# Autodesk Inventor assembly: 1000_Planar Winding Jig Overall Assembly_V1
(part 2 of 2)
- Mate:124: 1322_Clamp Holder_V1:2 ↔ 1323_Clamp Holder Pin_V1:2
- Mate:125: 1322_Clamp Holder_V1:1 ↔ 1323_Clamp Holder Pin_V1:1
- Angle:9 (0 deg): frame_1385mm:4 ↔ 1313_Former Bottom_V1:1
- Flush:135 (45 mm): 1324_Clamp Rail_V1:2 ↔ 1322_Clamp Holder_V1:2
- [Flush] (45 mm): 1324_Clamp Rail_V1:3 ↔ 1322_Clamp Holder_V1:3
- [Mate] (0.5 mm): 1324_Clamp Rail_V1:4 ↔ 1322_Clamp Holder_V1:3
- [Mate]: 1322_Clamp Holder_V1:3 ↔ 1321_Toggle Clamp_V1:3
- [Flush]: 1322_Clamp Holder_V1:3 ↔ 1321_Toggle Clamp_V1:3
- [Flush] (3 mm): 1322_Clamp Holder_V1:3 ↔ 1321_Toggle Clamp_V1:3
- [Mate]: 1322_Clamp Holder_V1:3 ↔ BS 3692 Precision hexagon bolts and screws (Full Threaded) - Metric M4 x 9:10
- [Mate]: 1322_Clamp Holder_V1:3 ↔ BS 3692 Precision hexagon bolts and screws (Full Threaded) - Metric M4 x 9:10
- [Angle] (0 deg): 1322_Clamp Holder_V1:3 ↔ BS 3692 Precision hexagon bolts and screws (Full Threaded) - Metric M4 x 9:10
- [Mate]: 1322_Clamp Holder_V1:3 ↔ BS 3692 Precision hexagon bolts and screws (Full Threaded) - Metric M4 x 9:9
- [Mate]: 1322_Clamp Holder_V1:3 ↔ BS 3692 Precision hexagon bolts and screws (Full Threaded) - Metric M4 x 9:9
- [Angle] (0 deg): 1322_Clamp Holder_V1:3 ↔ BS 3692 Precision hexagon bolts and screws (Full Threaded) - Metric M4 x 9:9
- [Flush]: BS 3692 Precision hexagon bolts and screws (Full Threaded) - Metric M4 x 9:11 ↔ BS 3692 Precision hexagon bolts and screws (Full Threaded) - Metric M4 x 9:12
- [Mate]: 1322_Clamp Holder_V1:3 ↔ BS 3692 Precision hexagon bolts and screws (Full Threaded) - Metric M4 x 9:12
- [Mate]: 1322_Clamp Holder_V1:3 ↔ BS 3692 Precision hexagon bolts and screws (Full Threaded) - Metric M4 x 9:12
- [Flush]: BS 3692 Precision hexagon bolts and screws (Full Threaded) - Metric M4 x 9:9 ↔ BS 3692 Precision hexagon bolts and screws (Full Threaded) - Metric M4 x 9:12
- [Mate]: 1322_Clamp Holder_V1:3 ↔ BS 3692 Precision hexagon bolts and screws (Full Threaded) - Metric M4 x 9:11
- [Flush]: BS 3692 Precision hexagon bolts and screws (Full Threaded) - Metric M4 x 9:10 ↔ BS 3692 Precision hexagon bolts and screws (Full Threaded) - Metric M4 x 9:11
- [Mate]: BS 3692 Precision hexagon bolts and screws (Full Threaded) - Metric M4 x 9:9 ↔ AS 1474 - Metric M4:9
- [Mate]: 1321_Toggle Clamp_V1:3 ↔ AS 1474 - Metric M4:9
- [Flush]: AS 1474 - Metric M4:10 ↔ AS 1474 - Metric M4:12
- [Flush]: AS 1474 - Metric M4:11 ↔ AS 1474 - Metric M4:12
- [Flush]: AS 1474 - Metric M4:10 ↔ AS 1474 - Metric M4:11
- [Mate]: BS 3692 Precision hexagon bolts and screws (Full Threaded) - Metric M4 x 9:12 ↔ AS 1474 - Metric M4:10
- [Mate]: 1321_Toggle Clamp_V1:3 ↔ AS 1474 - Metric M4:10
- [Mate]: BS 3692 Precision hexagon bolts and screws (Full Threaded) - Metric M4 x 9:11 ↔ AS 1474 - Metric M4:11
- [Mate]: 1321_Toggle Clamp_V1:3 ↔ AS 1474 - Metric M4:12
- [Mate]: BS 3692 Precision hexagon bolts and screws (Full Threaded) - Metric M4 x 9:10 ↔ AS 1474 - Metric M4:12
- [Flush]: AS 1474 - Metric M4:9 ↔ AS 1474 - Metric M4:12
- [Mate]: 1322_Clamp Holder_V1:4 ↔ 1321_Toggle Clamp_V1:4
- [Flush]: 1322_Clamp Holder_V1:4 ↔ 1321_Toggle Clamp_V1:4
- [Flush] (3 mm): 1322_Clamp Holder_V1:4 ↔ 1321_Toggle Clamp_V1:4
- [Mate]: 1322_Clamp Holder_V1:4 ↔ BS 3692 Precision hexagon bolts and screws (Full Threaded) - Metric M4 x 9:14
- [Mate]: 1322_Clamp Holder_V1:4 ↔ BS 3692 Precision hexagon bolts and screws (Full Threaded) - Metric M4 x 9:14
- [Angle] (0 deg): 1322_Clamp Holder_V1:4 ↔ BS 3692 Precision hexagon bolts and screws (Full Threaded) - Metric M4 x 9:14
- [Mate]: 1322_Clamp Holder_V1:4 ↔ BS 3692 Precision hexagon bolts and screws (Full Threaded) - Metric M4 x 9:13
- [Mate]: 1322_Clamp Holder_V1:4 ↔ BS 3692 Precision hexagon bolts and screws (Full Threaded) - Metric M4 x 9:13
- [Angle] (0 deg): 1322_Clamp Holder_V1:4 ↔ BS 3692 Precision hexagon bolts and screws (Full Threaded) - Metric M4 x 9:13
- [Flush]: BS 3692 Precision hexagon bolts and screws (Full Threaded) - Metric M4 x 9:15 ↔ BS 3692 Precision hexagon bolts and screws (Full Threaded) - Metric M4 x 9:16
- [Mate]: 1322_Clamp Holder_V1:4 ↔ BS 3692 Precision hexagon bolts and screws (Full Threaded) - Metric M4 x 9:16
- [Mate]: 1322_Clamp Holder_V1:4 ↔ BS 3692 Precision hexagon bolts and screws (Full Threaded) - Metric M4 x 9:16
- [Flush]: BS 3692 Precision hexagon bolts and screws (Full Threaded) - Metric M4 x 9:13 ↔ BS 3692 Precision hexagon bolts and screws (Full Threaded) - Metric M4 x 9:16
- [Mate]: 1322_Clamp Holder_V1:4 ↔ BS 3692 Precision hexagon bolts and screws (Full Threaded) - Metric M4 x 9:15
- [Flush]: BS 3692 Precision hexagon bolts and screws (Full Threaded) - Metric M4 x 9:14 ↔ BS 3692 Precision hexagon bolts and screws (Full Threaded) - Metric M4 x 9:15
- [Mate]: BS 3692 Precision hexagon bolts and screws (Full Threaded) - Metric M4 x 9:13 ↔ AS 1474 - Metric M4:13
- [Mate]: 1321_Toggle Clamp_V1:4 ↔ AS 1474 - Metric M4:13
- [Flush]: AS 1474 - Metric M4:14 ↔ AS 1474 - Metric M4:16
- [Flush]: AS 1474 - Metric M4:15 ↔ AS 1474 - Metric M4:16
- [Flush]: AS 1474 - Metric M4:14 ↔ AS 1474 - Metric M4:15
- [Mate]: BS 3692 Precision hexagon bolts and screws (Full Threaded) - Metric M4 x 9:16 ↔ AS 1474 - Metric M4:14
- [Mate]: 1321_Toggle Clamp_V1:4 ↔ AS 1474 - Metric M4:14
- [Mate]: BS 3692 Precision hexagon bolts and screws (Full Threaded) - Metric M4 x 9:15 ↔ AS 1474 - Metric M4:15
- [Mate]: 1321_Toggle Clamp_V1:4 ↔ AS 1474 - Metric M4:16
- [Mate]: BS 3692 Precision hexagon bolts and screws (Full Threaded) - Metric M4 x 9:14 ↔ AS 1474 - Metric M4:16
- [Flush]: AS 1474 - Metric M4:13 ↔ AS 1474 - Metric M4:16
- [Mate]: 1324_Clamp Rail_V1:4 ↔ 1322_Clamp Holder_V1:4
- [Mate]: 1322_Clamp Holder_V1:4 ↔ 1323_Clamp Holder Pin_V1:4
- [Mate]: 1322_Clamp Holder_V1:3 ↔ 1323_Clamp Holder Pin_V1:3
- [Flush] (45 mm): 1324_Clamp Rail_V1:4 ↔ 1322_Clamp Holder_V1:4
- Mate:160: 1311_Former Top_V1:1 ↔ 1324_Clamp Rail_V1:3
- Flush:156: 1324_Clamp Rail_V1:3 ↔ 1324_Clamp Rail_V1:4
- Mate:161: 1324_Clamp Rail_V1:4 ↔ 1322_Clamp Holder_V1:3
- Flush:157: 1322_Clamp Holder_V1:3 ↔ 1322_Clamp Holder_V1:4
- Mate:162: 1324_Clamp Rail_V1:3 ↔ 1322_Clamp Holder_V1:4
- Mate:163: 1311_Former Top_V1:1 ↔ 1324_Clamp Rail_V1:4
- Mate:164: 1311_Former Top_V1:1 ↔ 1324_Clamp Rail_V1:4
- Flush:158: 1324_Clamp Rail_V1:3 ↔ 1324_Clamp Rail_V1:4
- Flush:159: 1323_Clamp Holder Pin_V1:3 ↔ 1323_Clamp Holder Pin_V1:4
- Flush:160: 1311_Former Top_V1:1 ↔ 1323_Clamp Holder Pin_V1:4
- [Flush] (45 mm): 1324_Clamp Rail_V1:5 ↔ 1322_Clamp Holder_V1:5
- [Mate] (0.5 mm): 1324_Clamp Rail_V1:6 ↔ 1322_Clamp Holder_V1:5
- [Mate]: 1322_Clamp Holder_V1:5 ↔ 1321_Toggle Clamp_V1:5
- [Flush]: 1322_Clamp Holder_V1:5 ↔ 1321_Toggle Clamp_V1:5
- [Flush] (3 mm): 1322_Clamp Holder_V1:5 ↔ 1321_Toggle Clamp_V1:5
- [Mate]: 1322_Clamp Holder_V1:5 ↔ BS 3692 Precision hexagon bolts and screws (Full Threaded) - Metric M4 x 9:18
- [Mate]: 1322_Clamp Holder_V1:5 ↔ BS 3692 Precision hexagon bolts and screws (Full Threaded) - Metric M4 x 9:18
- [Angle] (0 deg): 1322_Clamp Holder_V1:5 ↔ BS 3692 Precision hexagon bolts and screws (Full Threaded) - Metric M4 x 9:18
- [Mate]: 1322_Clamp Holder_V1:5 ↔ BS 3692 Precision hexagon bolts and screws (Full Threaded) - Metric M4 x 9:17
- [Mate]: 1322_Clamp Holder_V1:5 ↔ BS 3692 Precision hexagon bolts and screws (Full Threaded) - Metric M4 x 9:17
- [Angle] (0 deg): 1322_Clamp Holder_V1:5 ↔ BS 3692 Precision hexagon bolts and screws (Full Threaded) - Metric M4 x 9:17
- [Flush]: BS 3692 Precision hexagon bolts and screws (Full Threaded) - Metric M4 x 9:19 ↔ BS 3692 Precision hexagon bolts and screws (Full Threaded) - Metric M4 x 9:20
- [Mate]: 1322_Clamp Holder_V1:5 ↔ BS 3692 Precision hexagon bolts and screws (Full Threaded) - Metric M4 x 9:20
- [Mate]: 1322_Clamp Holder_V1:5 ↔ BS 3692 Precision hexagon bolts and screws (Full Threaded) - Metric M4 x 9:20
- [Flush]: BS 3692 Precision hexagon bolts and screws (Full Threaded) - Metric M4 x 9:17 ↔ BS 3692 Precision hexagon bolts and screws (Full Threaded) - Metric M4 x 9:20
- [Mate]: 1322_Clamp Holder_V1:5 ↔ BS 3692 Precision hexagon bolts and screws (Full Threaded) - Metric M4 x 9:19
- [Flush]: BS 3692 Precision hexagon bolts and screws (Full Threaded) - Metric M4 x 9:18 ↔ BS 3692 Precision hexagon bolts and screws (Full Threaded) - Metric M4 x 9:19
- [Mate]: BS 3692 Precision hexagon bolts and screws (Full Threaded) - Metric M4 x 9:17 ↔ AS 1474 - Metric M4:17
- [Mate]: 1321_Toggle Clamp_V1:5 ↔ AS 1474 - Metric M4:17
- [Flush]: AS 1474 - Metric M4:18 ↔ AS 1474 - Metric M4:20
- [Flush]: AS 1474 - Metric M4:19 ↔ AS 1474 - Metric M4:20
- [Flush]: AS 1474 - Metric M4:18 ↔ AS 1474 - Metric M4:19
- [Mate]: BS 3692 Precision hexagon bolts and screws (Full Threaded) - Metric M4 x 9:20 ↔ AS 1474 - Metric M4:18
- [Mate]: 1321_Toggle Clamp_V1:5 ↔ AS 1474 - Metric M4:18
- [Mate]: BS 3692 Precision hexagon bolts and screws (Full Threaded) - Metric M4 x 9:19 ↔ AS 1474 - Metric M4:19
- [Mate]: 1321_Toggle Clamp_V1:5 ↔ AS 1474 - Metric M4:20
- [Mate]: BS 3692 Precision hexagon bolts and screws (Full Threaded) - Metric M4 x 9:18 ↔ AS 1474 - Metric M4:20
- [Flush]: AS 1474 - Metric M4:17 ↔ AS 1474 - Metric M4:20
- [Mate]: 1322_Clamp Holder_V1:6 ↔ 1321_Toggle Clamp_V1:6
- [Flush]: 1322_Clamp Holder_V1:6 ↔ 1321_Toggle Clamp_V1:6
- [Flush] (3 mm): 1322_Clamp Holder_V1:6 ↔ 1321_Toggle Clamp_V1:6
- [Mate]: 1322_Clamp Holder_V1:6 ↔ BS 3692 Precision hexagon bolts and screws (Full Threaded) - Metric M4 x 9:22
- [Mate]: 1322_Clamp Holder_V1:6 ↔ BS 3692 Precision hexagon bolts and screws (Full Threaded) - Metric M4 x 9:22
- [Angle] (0 deg): 1322_Clamp Holder_V1:6 ↔ BS 3692 Precision hexagon bolts and screws (Full Threaded) - Metric M4 x 9:22
- [Mate]: 1322_Clamp Holder_V1:6 ↔ BS 3692 Precision hexagon bolts and screws (Full Threaded) - Metric M4 x 9:21
- [Mate]: 1322_Clamp Holder_V1:6 ↔ BS 3692 Precision hexagon bolts and screws (Full Threaded) - Metric M4 x 9:21
- [Angle] (0 deg): 1322_Clamp Holder_V1:6 ↔ BS 3692 Precision hexagon bolts and screws (Full Threaded) - Metric M4 x 9:21
- [Flush]: BS 3692 Precision hexagon bolts and screws (Full Threaded) - Metric M4 x 9:23 ↔ BS 3692 Precision hexagon bolts and screws (Full Threaded) - Metric M4 x 9:24
- [Mate]: 1322_Clamp Holder_V1:6 ↔ BS 3692 Precision hexagon bolts and screws (Full Threaded) - Metric M4 x 9:24
- [Mate]: 1322_Clamp Holder_V1:6 ↔ BS 3692 Precision hexagon bolts and screws (Full Threaded) - Metric M4 x 9:24
- [Flush]: BS 3692 Precision hexagon bolts and screws (Full Threaded) - Metric M4 x 9:21 ↔ BS 3692 Precision hexagon bolts and screws (Full Threaded) - Metric M4 x 9:24
- [Mate]: 1322_Clamp Holder_V1:6 ↔ BS 3692 Precision hexagon bolts and screws (Full Threaded) - Metric M4 x 9:23
- [Flush]: BS 3692 Precision hexagon bolts and screws (Full Threaded) - Metric M4 x 9:22 ↔ BS 3692 Precision hexagon bolts and screws (Full Threaded) - Metric M4 x 9:23
- [Mate]: BS 3692 Precision hexagon bolts and screws (Full Threaded) - Metric M4 x 9:21 ↔ AS 1474 - Metric M4:21
- [Mate]: 1321_Toggle Clamp_V1:6 ↔ AS 1474 - Metric M4:21
- [Flush]: AS 1474 - Metric M4:22 ↔ AS 1474 - Metric M4:24
- [Flush]: AS 1474 - Metric M4:23 ↔ AS 1474 - Metric M4:24
- [Flush]: AS 1474 - Metric M4:22 ↔ AS 1474 - Metric M4:23
- [Mate]: BS 3692 Precision hexagon bolts and screws (Full Threaded) - Metric M4 x 9:24 ↔ AS 1474 - Metric M4:22
- [Mate]: 1321_Toggle Clamp_V1:6 ↔ AS 1474 - Metric M4:22
- [Mate]: BS 3692 Precision hexagon bolts and screws (Full Threaded) - Metric M4 x 9:23 ↔ AS 1474 - Metric M4:23
- [Mate]: 1321_Toggle Clamp_V1:6 ↔ AS 1474 - Metric M4:24
- [Mate]: BS 3692 Precision hexagon bolts and screws (Full Threaded) - Metric M4 x 9:22 ↔ AS 1474 - Metric M4:24
- [Flush]: AS 1474 - Metric M4:21 ↔ AS 1474 - Metric M4:24
- [Mate]: 1324_Clamp Rail_V1:6 ↔ 1322_Clamp Holder_V1:6
- [Mate]: 1322_Clamp Holder_V1:6 ↔ 1323_Clamp Holder Pin_V1:6
- [Mate]: 1322_Clamp Holder_V1:5 ↔ 1323_Clamp Holder Pin_V1:5
- [Flush] (45 mm): 1324_Clamp Rail_V1:6 ↔ 1322_Clamp Holder_V1:6
- [Flush]: 1324_Clamp Rail_V1:5 ↔ 1324_Clamp Rail_V1:6
- [Mate]: 1324_Clamp Rail_V1:6 ↔ 1322_Clamp Holder_V1:5
- [Flush]: 1322_Clamp Holder_V1:5 ↔ 1322_Clamp Holder_V1:6
- [Mate]: 1324_Clamp Rail_V1:5 ↔ 1322_Clamp Holder_V1:6
- [Flush]: 1324_Clamp Rail_V1:5 ↔ 1324_Clamp Rail_V1:6
- [Flush]: 1323_Clamp Holder Pin_V1:5 ↔ 1323_Clamp Holder Pin_V1:6
- Mate:201: 1311_Former Top_V1:1 ↔ 1324_Clamp Rail_V1:6
- Mate:202: 1311_Former Top_V1:1 ↔ 1324_Clamp Rail_V1:6
- Mate:203: 1311_Former Top_V1:1 ↔ 1324_Clamp Rail_V1:6
- Flush:185: 1323_Clamp Holder Pin_V1:2 ↔ 1323_Clamp Holder Pin_V1:6
- [Flush] (45 mm): 1324_Clamp Rail_V1:7 ↔ 1322_Clamp Holder_V1:7
- [Mate] (0.5 mm): 1324_Clamp Rail_V1:8 ↔ 1322_Clamp Holder_V1:7
- [Mate]: 1322_Clamp Holder_V1:7 ↔ 1321_Toggle Clamp_V1:7
- [Flush]: 1322_Clamp Holder_V1:7 ↔ 1321_Toggle Clamp_V1:7
- [Flush] (3 mm): 1322_Clamp Holder_V1:7 ↔ 1321_Toggle Clamp_V1:7
- [Mate]: 1322_Clamp Holder_V1:7 ↔ BS 3692 Precision hexagon bolts and screws (Full Threaded) - Metric M4 x 9:26
- [Mate]: 1322_Clamp Holder_V1:7 ↔ BS 3692 Precision hexagon bolts and screws (Full Threaded) - Metric M4 x 9:26
- [Angle] (0 deg): 1322_Clamp Holder_V1:7 ↔ BS 3692 Precision hexagon bolts and screws (Full Threaded) - Metric M4 x 9:26
- [Mate]: 1322_Clamp Holder_V1:7 ↔ BS 3692 Precision hexagon bolts and screws (Full Threaded) - Metric M4 x 9:25
- [Mate]: 1322_Clamp Holder_V1:7 ↔ BS 3692 Precision hexagon bolts and screws (Full Threaded) - Metric M4 x 9:25
- [Angle] (0 deg): 1322_Clamp Holder_V1:7 ↔ BS 3692 Precision hexagon bolts and screws (Full Threaded) - Metric M4 x 9:25
- [Flush]: BS 3692 Precision hexagon bolts and screws (Full Threaded) - Metric M4 x 9:27 ↔ BS 3692 Precision hexagon bolts and screws (Full Threaded) - Metric M4 x 9:28
- [Mate]: 1322_Clamp Holder_V1:7 ↔ BS 3692 Precision hexagon bolts and screws (Full Threaded) - Metric M4 x 9:28
- [Mate]: 1322_Clamp Holder_V1:7 ↔ BS 3692 Precision hexagon bolts and screws (Full Threaded) - Metric M4 x 9:28
- [Flush]: BS 3692 Precision hexagon bolts and screws (Full Threaded) - Metric M4 x 9:25 ↔ BS 3692 Precision hexagon bolts and screws (Full Threaded) - Metric M4 x 9:28
- [Mate]: 1322_Clamp Holder_V1:7 ↔ BS 3692 Precision hexagon bolts and screws (Full Threaded) - Metric M4 x 9:27
- [Flush]: BS 3692 Precision hexagon bolts and screws (Full Threaded) - Metric M4 x 9:26 ↔ BS 3692 Precision hexagon bolts and screws (Full Threaded) - Metric M4 x 9:27
- [Mate]: BS 3692 Precision hexagon bolts and screws (Full Threaded) - Metric M4 x 9:25 ↔ AS 1474 - Metric M4:25
- [Mate]: 1321_Toggle Clamp_V1:7 ↔ AS 1474 - Metric M4:25
- [Flush]: AS 1474 - Metric M4:26 ↔ AS 1474 - Metric M4:28
- [Flush]: AS 1474 - Metric M4:27 ↔ AS 1474 - Metric M4:28
- [Flush]: AS 1474 - Metric M4:26 ↔ AS 1474 - Metric M4:27
- [Mate]: BS 3692 Precision hexagon bolts and screws (Full Threaded) - Metric M4 x 9:28 ↔ AS 1474 - Metric M4:26
- [Mate]: 1321_Toggle Clamp_V1:7 ↔ AS 1474 - Metric M4:26
- [Mate]: BS 3692 Precision hexagon bolts and screws (Full Threaded) - Metric M4 x 9:27 ↔ AS 1474 - Metric M4:27
- [Mate]: 1321_Toggle Clamp_V1:7 ↔ AS 1474 - Metric M4:28
- [Mate]: BS 3692 Precision hexagon bolts and screws (Full Threaded) - Metric M4 x 9:26 ↔ AS 1474 - Metric M4:28
- [Flush]: AS 1474 - Metric M4:25 ↔ AS 1474 - Metric M4:28
- [Mate]: 1322_Clamp Holder_V1:8 ↔ 1321_Toggle Clamp_V1:8
- [Flush]: 1322_Clamp Holder_V1:8 ↔ 1321_Toggle Clamp_V1:8
- [Flush] (3 mm): 1322_Clamp Holder_V1:8 ↔ 1321_Toggle Clamp_V1:8
- [Mate]: 1322_Clamp Holder_V1:8 ↔ BS 3692 Precision hexagon bolts and screws (Full Threaded) - Metric M4 x 9:30
- [Mate]: 1322_Clamp Holder_V1:8 ↔ BS 3692 Precision hexagon bolts and screws (Full Threaded) - Metric M4 x 9:30
- [Angle] (0 deg): 1322_Clamp Holder_V1:8 ↔ BS 3692 Precision hexagon bolts and screws (Full Threaded) - Metric M4 x 9:30
- [Mate]: 1322_Clamp Holder_V1:8 ↔ BS 3692 Precision hexagon bolts and screws (Full Threaded) - Metric M4 x 9:29
- [Mate]: 1322_Clamp Holder_V1:8 ↔ BS 3692 Precision hexagon bolts and screws (Full Threaded) - Metric M4 x 9:29
- [Angle] (0 deg): 1322_Clamp Holder_V1:8 ↔ BS 3692 Precision hexagon bolts and screws (Full Threaded) - Metric M4 x 9:29
- [Flush]: BS 3692 Precision hexagon bolts and screws (Full Threaded) - Metric M4 x 9:31 ↔ BS 3692 Precision hexagon bolts and screws (Full Threaded) - Metric M4 x 9:32
- [Mate]: 1322_Clamp Holder_V1:8 ↔ BS 3692 Precision hexagon bolts and screws (Full Threaded) - Metric M4 x 9:32
- [Mate]: 1322_Clamp Holder_V1:8 ↔ BS 3692 Precision hexagon bolts and screws (Full Threaded) - Metric M4 x 9:32
- [Flush]: BS 3692 Precision hexagon bolts and screws (Full Threaded) - Metric M4 x 9:29 ↔ BS 3692 Precision hexagon bolts and screws (Full Threaded) - Metric M4 x 9:32
- [Mate]: 1322_Clamp Holder_V1:8 ↔ BS 3692 Precision hexagon bolts and screws (Full Threaded) - Metric M4 x 9:31
- [Flush]: BS 3692 Precision hexagon bolts and screws (Full Threaded) - Metric M4 x 9:30 ↔ BS 3692 Precision hexagon bolts and screws (Full Threaded) - Metric M4 x 9:31
- [Mate]: BS 3692 Precision hexagon bolts and screws (Full Threaded) - Metric M4 x 9:29 ↔ AS 1474 - Metric M4:29
- [Mate]: 1321_Toggle Clamp_V1:8 ↔ AS 1474 - Metric M4:29
- [Flush]: AS 1474 - Metric M4:30 ↔ AS 1474 - Metric M4:32
- [Flush]: AS 1474 - Metric M4:31 ↔ AS 1474 - Metric M4:32
- [Flush]: AS 1474 - Metric M4:30 ↔ AS 1474 - Metric M4:31
- [Mate]: BS 3692 Precision hexagon bolts and screws (Full Threaded) - Metric M4 x 9:32 ↔ AS 1474 - Metric M4:30
- [Mate]: 1321_Toggle Clamp_V1:8 ↔ AS 1474 - Metric M4:30
- [Mate]: BS 3692 Precision hexagon bolts and screws (Full Threaded) - Metric M4 x 9:31 ↔ AS 1474 - Metric M4:31
- [Mate]: 1321_Toggle Clamp_V1:8 ↔ AS 1474 - Metric M4:32
- [Mate]: BS 3692 Precision hexagon bolts and screws (Full Threaded) - Metric M4 x 9:30 ↔ AS 1474 - Metric M4:32
- [Flush]: AS 1474 - Metric M4:29 ↔ AS 1474 - Metric M4:32
- [Mate]: 1324_Clamp Rail_V1:8 ↔ 1322_Clamp Holder_V1:8
- [Mate]: 1322_Clamp Holder_V1:8 ↔ 1323_Clamp Holder Pin_V1:8
- [Mate]: 1322_Clamp Holder_V1:7 ↔ 1323_Clamp Holder Pin_V1:7
- [Flush] (45 mm): 1324_Clamp Rail_V1:8 ↔ 1322_Clamp Holder_V1:8
- [Flush]: 1324_Clamp Rail_V1:7 ↔ 1324_Clamp Rail_V1:8
- [Mate]: 1324_Clamp Rail_V1:8 ↔ 1322_Clamp Holder_V1:7
- [Flush]: 1322_Clamp Holder_V1:7 ↔ 1322_Clamp Holder_V1:8
- [Mate]: 1324_Clamp Rail_V1:7 ↔ 1322_Clamp Holder_V1:8
- [Flush]: 1324_Clamp Rail_V1:7 ↔ 1324_Clamp Rail_V1:8
- [Flush]: 1323_Clamp Holder Pin_V1:7 ↔ 1323_Clamp Holder Pin_V1:8
- [Flush] (45 mm): 1324_Clamp Rail_V1:9 ↔ 1322_Clamp Holder_V1:9
- [Mate] (0.5 mm): 1324_Clamp Rail_V1:10 ↔ 1322_Clamp Holder_V1:9
- [Mate]: 1322_Clamp Holder_V1:9 ↔ 1321_Toggle Clamp_V1:9
- [Flush]: 1322_Clamp Holder_V1:9 ↔ 1321_Toggle Clamp_V1:9
- [Flush] (3 mm): 1322_Clamp Holder_V1:9 ↔ 1321_Toggle Clamp_V1:9
- [Mate]: 1322_Clamp Holder_V1:9 ↔ BS 3692 Precision hexagon bolts and screws (Full Threaded) - Metric M4 x 9:34
- [Mate]: 1322_Clamp Holder_V1:9 ↔ BS 3692 Precision hexagon bolts and screws (Full Threaded) - Metric M4 x 9:34
- [Angle] (0 deg): 1322_Clamp Holder_V1:9 ↔ BS 3692 Precision hexagon bolts and screws (Full Threaded) - Metric M4 x 9:34
- [Mate]: 1322_Clamp Holder_V1:9 ↔ BS 3692 Precision hexagon bolts and screws (Full Threaded) - Metric M4 x 9:33
- [Mate]: 1322_Clamp Holder_V1:9 ↔ BS 3692 Precision hexagon bolts and screws (Full Threaded) - Metric M4 x 9:33
- [Angle] (0 deg): 1322_Clamp Holder_V1:9 ↔ BS 3692 Precision hexagon bolts and screws (Full Threaded) - Metric M4 x 9:33
- [Flush]: BS 3692 Precision hexagon bolts and screws (Full Threaded) - Metric M4 x 9:35 ↔ BS 3692 Precision hexagon bolts and screws (Full Threaded) - Metric M4 x 9:36
- [Mate]: 1322_Clamp Holder_V1:9 ↔ BS 3692 Precision hexagon bolts and screws (Full Threaded) - Metric M4 x 9:36
- [Mate]: 1322_Clamp Holder_V1:9 ↔ BS 3692 Precision hexagon bolts and screws (Full Threaded) - Metric M4 x 9:36
- [Flush]: BS 3692 Precision hexagon bolts and screws (Full Threaded) - Metric M4 x 9:33 ↔ BS 3692 Precision hexagon bolts and screws (Full Threaded) - Metric M4 x 9:36
- [Mate]: 1322_Clamp Holder_V1:9 ↔ BS 3692 Precision hexagon bolts and screws (Full Threaded) - Metric M4 x 9:35
- [Flush]: BS 3692 Precision hexagon bolts and screws (Full Threaded) - Metric M4 x 9:34 ↔ BS 3692 Precision hexagon bolts and screws (Full Threaded) - Metric M4 x 9:35
- [Mate]: BS 3692 Precision hexagon bolts and screws (Full Threaded) - Metric M4 x 9:33 ↔ AS 1474 - Metric M4:33
- [Mate]: 1321_Toggle Clamp_V1:9 ↔ AS 1474 - Metric M4:33
- [Flush]: AS 1474 - Metric M4:34 ↔ AS 1474 - Metric M4:36
- [Flush]: AS 1474 - Metric M4:35 ↔ AS 1474 - Metric M4:36
- [Flush]: AS 1474 - Metric M4:34 ↔ AS 1474 - Metric M4:35
- [Mate]: BS 3692 Precision hexagon bolts and screws (Full Threaded) - Metric M4 x 9:36 ↔ AS 1474 - Metric M4:34
- [Mate]: 1321_Toggle Clamp_V1:9 ↔ AS 1474 - Metric M4:34
- [Mate]: BS 3692 Precision hexagon bolts and screws (Full Threaded) - Metric M4 x 9:35 ↔ AS 1474 - Metric M4:35
- [Mate]: 1321_Toggle Clamp_V1:9 ↔ AS 1474 - Metric M4:36
- [Mate]: BS 3692 Precision hexagon bolts and screws (Full Threaded) - Metric M4 x 9:34 ↔ AS 1474 - Metric M4:36
- [Flush]: AS 1474 - Metric M4:33 ↔ AS 1474 - Metric M4:36
- [Mate]: 1322_Clamp Holder_V1:10 ↔ 1321_Toggle Clamp_V1:10
- [Flush]: 1322_Clamp Holder_V1:10 ↔ 1321_Toggle Clamp_V1:10
- [Flush] (3 mm): 1322_Clamp Holder_V1:10 ↔ 1321_Toggle Clamp_V1:10
- [Mate]: 1322_Clamp Holder_V1:10 ↔ BS 3692 Precision hexagon bolts and screws (Full Threaded) - Metric M4 x 9:38
- [Mate]: 1322_Clamp Holder_V1:10 ↔ BS 3692 Precision hexagon bolts and screws (Full Threaded) - Metric M4 x 9:38
- [Angle] (0 deg): 1322_Clamp Holder_V1:10 ↔ BS 3692 Precision hexagon bolts and screws (Full Threaded) - Metric M4 x 9:38
- [Mate]: 1322_Clamp Holder_V1:10 ↔ BS 3692 Precision hexagon bolts and screws (Full Threaded) - Metric M4 x 9:37
- [Mate]: 1322_Clamp Holder_V1:10 ↔ BS 3692 Precision hexagon bolts and screws (Full Threaded) - Metric M4 x 9:37
- [Angle] (0 deg): 1322_Clamp Holder_V1:10 ↔ BS 3692 Precision hexagon bolts and screws (Full Threaded) - Metric M4 x 9:37
- [Flush]: BS 3692 Precision hexagon bolts and screws (Full Threaded) - Metric M4 x 9:39 ↔ BS 3692 Precision hexagon bolts and screws (Full Threaded) - Metric M4 x 9:40
- [Mate]: 1322_Clamp Holder_V1:10 ↔ BS 3692 Precision hexagon bolts and screws (Full Threaded) - Metric M4 x 9:40
- [Mate]: 1322_Clamp Holder_V1:10 ↔ BS 3692 Precision hexagon bolts and screws (Full Threaded) - Metric M4 x 9:40
- [Flush]: BS 3692 Precision hexagon bolts and screws (Full Threaded) - Metric M4 x 9:37 ↔ BS 3692 Precision hexagon bolts and screws (Full Threaded) - Metric M4 x 9:40
- [Mate]: 1322_Clamp Holder_V1:10 ↔ BS 3692 Precision hexagon bolts and screws (Full Threaded) - Metric M4 x 9:39
- [Flush]: BS 3692 Precision hexagon bolts and screws (Full Threaded) - Metric M4 x 9:38 ↔ BS 3692 Precision hexagon bolts and screws (Full Threaded) - Metric M4 x 9:39
- [Mate]: BS 3692 Precision hexagon bolts and screws (Full Threaded) - Metric M4 x 9:37 ↔ AS 1474 - Metric M4:37
- [Mate]: 1321_Toggle Clamp_V1:10 ↔ AS 1474 - Metric M4:37
- [Flush]: AS 1474 - Metric M4:38 ↔ AS 1474 - Metric M4:40
- [Flush]: AS 1474 - Metric M4:39 ↔ AS 1474 - Metric M4:40
- [Flush]: AS 1474 - Metric M4:38 ↔ AS 1474 - Metric M4:39
- [Mate]: BS 3692 Precision hexagon bolts and screws (Full Threaded) - Metric M4 x 9:40 ↔ AS 1474 - Metric M4:38
- [Mate]: 1321_Toggle Clamp_V1:10 ↔ AS 1474 - Metric M4:38
- [Mate]: BS 3692 Precision hexagon bolts and screws (Full Threaded) - Metric M4 x 9:39 ↔ AS 1474 - Metric M4:39
- [Mate]: 1321_Toggle Clamp_V1:10 ↔ AS 1474 - Metric M4:40
- [Mate]: BS 3692 Precision hexagon bolts and screws (Full Threaded) - Metric M4 x 9:38 ↔ AS 1474 - Metric M4:40
- [Flush]: AS 1474 - Metric M4:37 ↔ AS 1474 - Metric M4:40
- [Mate]: 1324_Clamp Rail_V1:10 ↔ 1322_Clamp Holder_V1:10
- [Mate]: 1322_Clamp Holder_V1:10 ↔ 1323_Clamp Holder Pin_V1:10
- [Mate]: 1322_Clamp Holder_V1:9 ↔ 1323_Clamp Holder Pin_V1:9
- [Flush] (45 mm): 1324_Clamp Rail_V1:10 ↔ 1322_Clamp Holder_V1:10
- [Flush]: 1324_Clamp Rail_V1:9 ↔ 1324_Clamp Rail_V1:10
- [Mate]: 1324_Clamp Rail_V1:10 ↔ 1322_Clamp Holder_V1:9
- [Flush]: 1322_Clamp Holder_V1:9 ↔ 1322_Clamp Holder_V1:10
- [Mate]: 1324_Clamp Rail_V1:9 ↔ 1322_Clamp Holder_V1:10
- [Flush]: 1324_Clamp Rail_V1:9 ↔ 1324_Clamp Rail_V1:10
- [Flush]: 1323_Clamp Holder Pin_V1:9 ↔ 1323_Clamp Holder Pin_V1:10
- [Flush] (45 mm): 1324_Clamp Rail_V1:11 ↔ 1322_Clamp Holder_V1:11
- [Mate] (0.5 mm): 1324_Clamp Rail_V1:12 ↔ 1322_Clamp Holder_V1:11
- [Mate]: 1322_Clamp Holder_V1:11 ↔ 1321_Toggle Clamp_V1:11
- [Flush]: 1322_Clamp Holder_V1:11 ↔ 1321_Toggle Clamp_V1:11
- [Flush] (3 mm): 1322_Clamp Holder_V1:11 ↔ 1321_Toggle Clamp_V1:11
- [Mate]: 1322_Clamp Holder_V1:11 ↔ BS 3692 Precision hexagon bolts and screws (Full Threaded) - Metric M4 x 9:42
- [Mate]: 1322_Clamp Holder_V1:11 ↔ BS 3692 Precision hexagon bolts and screws (Full Threaded) - Metric M4 x 9:42
- [Angle] (0 deg): 1322_Clamp Holder_V1:11 ↔ BS 3692 Precision hexagon bolts and screws (Full Threaded) - Metric M4 x 9:42
- [Mate]: 1322_Clamp Holder_V1:11 ↔ BS 3692 Precision hexagon bolts and screws (Full Threaded) - Metric M4 x 9:41
- [Mate]: 1322_Clamp Holder_V1:11 ↔ BS 3692 Precision hexagon bolts and screws (Full Threaded) - Metric M4 x 9:41
- [Angle] (0 deg): 1322_Clamp Holder_V1:11 ↔ BS 3692 Precision hexagon bolts and screws (Full Threaded) - Metric M4 x 9:41
- [Flush]: BS 3692 Precision hexagon bolts and screws (Full Threaded) - Metric M4 x 9:43 ↔ BS 3692 Precision hexagon bolts and screws (Full Threaded) - Metric M4 x 9:44
- [Mate]: 1322_Clamp Holder_V1:11 ↔ BS 3692 Precision hexagon bolts and screws (Full Threaded) - Metric M4 x 9:44
- [Mate]: 1322_Clamp Holder_V1:11 ↔ BS 3692 Precision hexagon bolts and screws (Full Threaded) - Metric M4 x 9:44
- [Flush]: BS 3692 Precision hexagon bolts and screws (Full Threaded) - Metric M4 x 9:41 ↔ BS 3692 Precision hexagon bolts and screws (Full Threaded) - Metric M4 x 9:44
- [Mate]: 1322_Clamp Holder_V1:11 ↔ BS 3692 Precision hexagon bolts and screws (Full Threaded) - Metric M4 x 9:43
- [Flush]: BS 3692 Precision hexagon bolts and screws (Full Threaded) - Metric M4 x 9:42 ↔ BS 3692 Precision hexagon bolts and screws (Full Threaded) - Metric M4 x 9:43
- [Mate]: BS 3692 Precision hexagon bolts and screws (Full Threaded) - Metric M4 x 9:41 ↔ AS 1474 - Metric M4:41
- [Mate]: 1321_Toggle Clamp_V1:11 ↔ AS 1474 - Metric M4:41
- [Flush]: AS 1474 - Metric M4:42 ↔ AS 1474 - Metric M4:44
- [Flush]: AS 1474 - Metric M4:43 ↔ AS 1474 - Metric M4:44
- [Flush]: AS 1474 - Metric M4:42 ↔ AS 1474 - Metric M4:43
- [Mate]: BS 3692 Precision hexagon bolts and screws (Full Threaded) - Metric M4 x 9:44 ↔ AS 1474 - Metric M4:42
- [Mate]: 1321_Toggle Clamp_V1:11 ↔ AS 1474 - Metric M4:42
- [Mate]: BS 3692 Precision hexagon bolts and screws (Full Threaded) - Metric M4 x 9:43 ↔ AS 1474 - Metric M4:43
- [Mate]: 1321_Toggle Clamp_V1:11 ↔ AS 1474 - Metric M4:44
- [Mate]: BS 3692 Precision hexagon bolts and screws (Full Threaded) - Metric M4 x 9:42 ↔ AS 1474 - Metric M4:44
- [Flush]: AS 1474 - Metric M4:41 ↔ AS 1474 - Metric M4:44
- [Mate]: 1322_Clamp Holder_V1:12 ↔ 1321_Toggle Clamp_V1:12
- [Flush]: 1322_Clamp Holder_V1:12 ↔ 1321_Toggle Clamp_V1:12
- [Flush] (3 mm): 1322_Clamp Holder_V1:12 ↔ 1321_Toggle Clamp_V1:12
- [Mate]: 1322_Clamp Holder_V1:12 ↔ BS 3692 Precision hexagon bolts and screws (Full Threaded) - Metric M4 x 9:46
- [Mate]: 1322_Clamp Holder_V1:12 ↔ BS 3692 Precision hexagon bolts and screws (Full Threaded) - Metric M4 x 9:46
- [Angle] (0 deg): 1322_Clamp Holder_V1:12 ↔ BS 3692 Precision hexagon bolts and screws (Full Threaded) - Metric M4 x 9:46
- [Mate]: 1322_Clamp Holder_V1:12 ↔ BS 3692 Precision hexagon bolts and screws (Full Threaded) - Metric M4 x 9:45
- [Mate]: 1322_Clamp Holder_V1:12 ↔ BS 3692 Precision hexagon bolts and screws (Full Threaded) - Metric M4 x 9:45
- [Angle] (0 deg): 1322_Clamp Holder_V1:12 ↔ BS 3692 Precision hexagon bolts and screws (Full Threaded) - Metric M4 x 9:45
- [Flush]: BS 3692 Precision hexagon bolts and screws (Full Threaded) - Metric M4 x 9:47 ↔ BS 3692 Precision hexagon bolts and screws (Full Threaded) - Metric M4 x 9:48
- [Mate]: 1322_Clamp Holder_V1:12 ↔ BS 3692 Precision hexagon bolts and screws (Full Threaded) - Metric M4 x 9:48
- [Mate]: 1322_Clamp Holder_V1:12 ↔ BS 3692 Precision hexagon bolts and screws (Full Threaded) - Metric M4 x 9:48
- [Flush]: BS 3692 Precision hexagon bolts and screws (Full Threaded) - Metric M4 x 9:45 ↔ BS 3692 Precision hexagon bolts and screws (Full Threaded) - Metric M4 x 9:48
- [Mate]: 1322_Clamp Holder_V1:12 ↔ BS 3692 Precision hexagon bolts and screws (Full Threaded) - Metric M4 x 9:47
- [Flush]: BS 3692 Precision hexagon bolts and screws (Full Threaded) - Metric M4 x 9:46 ↔ BS 3692 Precision hexagon bolts and screws (Full Threaded) - Metric M4 x 9:47
- [Mate]: BS 3692 Precision hexagon bolts and screws (Full Threaded) - Metric M4 x 9:45 ↔ AS 1474 - Metric M4:45
- [Mate]: 1321_Toggle Clamp_V1:12 ↔ AS 1474 - Metric M4:45
- [Flush]: AS 1474 - Metric M4:46 ↔ AS 1474 - Metric M4:48
- [Flush]: AS 1474 - Metric M4:47 ↔ AS 1474 - Metric M4:48
- [Flush]: AS 1474 - Metric M4:46 ↔ AS 1474 - Metric M4:47
- [Mate]: BS 3692 Precision hexagon bolts and screws (Full Threaded) - Metric M4 x 9:48 ↔ AS 1474 - Metric M4:46
- [Mate]: 1321_Toggle Clamp_V1:12 ↔ AS 1474 - Metric M4:46
- [Mate]: BS 3692 Precision hexagon bolts and screws (Full Threaded) - Metric M4 x 9:47 ↔ AS 1474 - Metric M4:47
- [Mate]: 1321_Toggle Clamp_V1:12 ↔ AS 1474 - Metric M4:48
- [Mate]: BS 3692 Precision hexagon bolts and screws (Full Threaded) - Metric M4 x 9:46 ↔ AS 1474 - Metric M4:48
- [Flush]: AS 1474 - Metric M4:45 ↔ AS 1474 - Metric M4:48
- [Mate]: 1324_Clamp Rail_V1:12 ↔ 1322_Clamp Holder_V1:12
- [Mate]: 1322_Clamp Holder_V1:12 ↔ 1323_Clamp Holder Pin_V1:12
- [Mate]: 1322_Clamp Holder_V1:11 ↔ 1323_Clamp Holder Pin_V1:11
- [Flush] (45 mm): 1324_Clamp Rail_V1:12 ↔ 1322_Clamp Holder_V1:12
- [Flush]: 1324_Clamp Rail_V1:11 ↔ 1324_Clamp Rail_V1:12
- [Mate]: 1324_Clamp Rail_V1:12 ↔ 1322_Clamp Holder_V1:11
- [Flush]: 1322_Clamp Holder_V1:11 ↔ 1322_Clamp Holder_V1:12
- [Mate]: 1324_Clamp Rail_V1:11 ↔ 1322_Clamp Holder_V1:12
- [Flush]: 1324_Clamp Rail_V1:11 ↔ 1324_Clamp Rail_V1:12
- [Flush]: 1323_Clamp Holder Pin_V1:11 ↔ 1323_Clamp Holder Pin_V1:12
- [Flush] (45 mm): 1324_Clamp Rail_V1:13 ↔ 1322_Clamp Holder_V1:13
- [Mate] (0.5 mm): 1324_Clamp Rail_V1:14 ↔ 1322_Clamp Holder_V1:13
- [Mate]: 1322_Clamp Holder_V1:13 ↔ 1321_Toggle Clamp_V1:13
- [Flush]: 1322_Clamp Holder_V1:13 ↔ 1321_Toggle Clamp_V1:13
- [Flush] (3 mm): 1322_Clamp Holder_V1:13 ↔ 1321_Toggle Clamp_V1:13
- [Mate]: 1322_Clamp Holder_V1:13 ↔ BS 3692 Precision hexagon bolts and screws (Full Threaded) - Metric M4 x 9:50
- [Mate]: 1322_Clamp Holder_V1:13 ↔ BS 3692 Precision hexagon bolts and screws (Full Threaded) - Metric M4 x 9:50
- [Angle] (0 deg): 1322_Clamp Holder_V1:13 ↔ BS 3692 Precision hexagon bolts and screws (Full Threaded) - Metric M4 x 9:50
- [Mate]: 1322_Clamp Holder_V1:13 ↔ BS 3692 Precision hexagon bolts and screws (Full Threaded) - Metric M4 x 9:49
- [Mate]: 1322_Clamp Holder_V1:13 ↔ BS 3692 Precision hexagon bolts and screws (Full Threaded) - Metric M4 x 9:49
- [Angle] (0 deg): 1322_Clamp Holder_V1:13 ↔ BS 3692 Precision hexagon bolts and screws (Full Threaded) - Metric M4 x 9:49
- [Flush]: BS 3692 Precision hexagon bolts and screws (Full Threaded) - Metric M4 x 9:51 ↔ BS 3692 Precision hexagon bolts and screws (Full Threaded) - Metric M4 x 9:52
- [Mate]: 1322_Clamp Holder_V1:13 ↔ BS 3692 Precision hexagon bolts and screws (Full Threaded) - Metric M4 x 9:52
- [Mate]: 1322_Clamp Holder_V1:13 ↔ BS 3692 Precision hexagon bolts and screws (Full Threaded) - Metric M4 x 9:52
- [Flush]: BS 3692 Precision hexagon bolts and screws (Full Threaded) - Metric M4 x 9:49 ↔ BS 3692 Precision hexagon bolts and screws (Full Threaded) - Metric M4 x 9:52
- [Mate]: 1322_Clamp Holder_V1:13 ↔ BS 3692 Precision hexagon bolts and screws (Full Threaded) - Metric M4 x 9:51
- [Flush]: BS 3692 Precision hexagon bolts and screws (Full Threaded) - Metric M4 x 9:50 ↔ BS 3692 Precision hexagon bolts and screws (Full Threaded) - Metric M4 x 9:51
- [Mate]: BS 3692 Precision hexagon bolts and screws (Full Threaded) - Metric M4 x 9:49 ↔ AS 1474 - Metric M4:49
- [Mate]: 1321_Toggle Clamp_V1:13 ↔ AS 1474 - Metric M4:49
- [Flush]: AS 1474 - Metric M4:50 ↔ AS 1474 - Metric M4:52
- [Flush]: AS 1474 - Metric M4:51 ↔ AS 1474 - Metric M4:52
- [Flush]: AS 1474 - Metric M4:50 ↔ AS 1474 - Metric M4:51
- [Mate]: BS 3692 Precision hexagon bolts and screws (Full Threaded) - Metric M4 x 9:52 ↔ AS 1474 - Metric M4:50
- [Mate]: 1321_Toggle Clamp_V1:13 ↔ AS 1474 - Metric M4:50
- [Mate]: BS 3692 Precision hexagon bolts and screws (Full Threaded) - Metric M4 x 9:51 ↔ AS 1474 - Metric M4:51
- [Mate]: 1321_Toggle Clamp_V1:13 ↔ AS 1474 - Metric M4:52
- [Mate]: BS 3692 Precision hexagon bolts and screws (Full Threaded) - Metric M4 x 9:50 ↔ AS 1474 - Metric M4:52
- [Flush]: AS 1474 - Metric M4:49 ↔ AS 1474 - Metric M4:52
- [Mate]: 1322_Clamp Holder_V1:14 ↔ 1321_Toggle Clamp_V1:14
- [Flush]: 1322_Clamp Holder_V1:14 ↔ 1321_Toggle Clamp_V1:14
- [Flush] (3 mm): 1322_Clamp Holder_V1:14 ↔ 1321_Toggle Clamp_V1:14
- [Mate]: 1322_Clamp Holder_V1:14 ↔ BS 3692 Precision hexagon bolts and screws (Full Threaded) - Metric M4 x 9:54
- [Mate]: 1322_Clamp Holder_V1:14 ↔ BS 3692 Precision hexagon bolts and screws (Full Threaded) - Metric M4 x 9:54
- [Angle] (0 deg): 1322_Clamp Holder_V1:14 ↔ BS 3692 Precision hexagon bolts and screws (Full Threaded) - Metric M4 x 9:54
- [Mate]: 1322_Clamp Holder_V1:14 ↔ BS 3692 Precision hexagon bolts and screws (Full Threaded) - Metric M4 x 9:53
- [Mate]: 1322_Clamp Holder_V1:14 ↔ BS 3692 Precision hexagon bolts and screws (Full Threaded) - Metric M4 x 9:53
- [Angle] (0 deg): 1322_Clamp Holder_V1:14 ↔ BS 3692 Precision hexagon bolts and screws (Full Threaded) - Metric M4 x 9:53
- [Flush]: BS 3692 Precision hexagon bolts and screws (Full Threaded) - Metric M4 x 9:55 ↔ BS 3692 Precision hexagon bolts and screws (Full Threaded) - Metric M4 x 9:56
- [Mate]: 1322_Clamp Holder_V1:14 ↔ BS 3692 Precision hexagon bolts and screws (Full Threaded) - Metric M4 x 9:56
- [Mate]: 1322_Clamp Holder_V1:14 ↔ BS 3692 Precision hexagon bolts and screws (Full Threaded) - Metric M4 x 9:56
- [Flush]: BS 3692 Precision hexagon bolts and screws (Full Threaded) - Metric M4 x 9:53 ↔ BS 3692 Precision hexagon bolts and screws (Full Threaded) - Metric M4 x 9:56
- [Mate]: 1322_Clamp Holder_V1:14 ↔ BS 3692 Precision hexagon bolts and screws (Full Threaded) - Metric M4 x 9:55
- [Flush]: BS 3692 Precision hexagon bolts and screws (Full Threaded) - Metric M4 x 9:54 ↔ BS 3692 Precision hexagon bolts and screws (Full Threaded) - Metric M4 x 9:55
- [Mate]: BS 3692 Precision hexagon bolts and screws (Full Threaded) - Metric M4 x 9:53 ↔ AS 1474 - Metric M4:53
- [Mate]: 1321_Toggle Clamp_V1:14 ↔ AS 1474 - Metric M4:53
- [Flush]: AS 1474 - Metric M4:54 ↔ AS 1474 - Metric M4:56
- [Flush]: AS 1474 - Metric M4:55 ↔ AS 1474 - Metric M4:56
- [Flush]: AS 1474 - Metric M4:54 ↔ AS 1474 - Metric M4:55
- [Mate]: BS 3692 Precision hexagon bolts and screws (Full Threaded) - Metric M4 x 9:56 ↔ AS 1474 - Metric M4:54
- [Mate]: 1321_Toggle Clamp_V1:14 ↔ AS 1474 - Metric M4:54
- [Mate]: BS 3692 Precision hexagon bolts and screws (Full Threaded) - Metric M4 x 9:55 ↔ AS 1474 - Metric M4:55
- [Mate]: 1321_Toggle Clamp_V1:14 ↔ AS 1474 - Metric M4:56
- [Mate]: BS 3692 Precision hexagon bolts and screws (Full Threaded) - Metric M4 x 9:54 ↔ AS 1474 - Metric M4:56
- [Flush]: AS 1474 - Metric M4:53 ↔ AS 1474 - Metric M4:56
- [Mate]: 1324_Clamp Rail_V1:14 ↔ 1322_Clamp Holder_V1:14
- [Mate]: 1322_Clamp Holder_V1:14 ↔ 1323_Clamp Holder Pin_V1:14
- [Mate]: 1322_Clamp Holder_V1:13 ↔ 1323_Clamp Holder Pin_V1:13
- [Flush] (45 mm): 1324_Clamp Rail_V1:14 ↔ 1322_Clamp Holder_V1:14
- [Flush]: 1324_Clamp Rail_V1:13 ↔ 1324_Clamp Rail_V1:14
- [Mate]: 1324_Clamp Rail_V1:14 ↔ 1322_Clamp Holder_V1:13
- [Flush]: 1322_Clamp Holder_V1:13 ↔ 1322_Clamp Holder_V1:14
- [Mate]: 1324_Clamp Rail_V1:13 ↔ 1322_Clamp Holder_V1:14
- [Flush]: 1324_Clamp Rail_V1:13 ↔ 1324_Clamp Rail_V1:14
- [Flush]: 1323_Clamp Holder Pin_V1:13 ↔ 1323_Clamp Holder Pin_V1:14
- Flush:282: 1324_Clamp Rail_V1:7 ↔ 1324_Clamp Rail_V1:10
- Flush:283: 1324_Clamp Rail_V1:10 ↔ 1324_Clamp Rail_V1:12
- Flush:284: 1324_Clamp Rail_V1:11 ↔ 1324_Clamp Rail_V1:14
- Flush:285: 1324_Clamp Rail_V1:7 ↔ 1324_Clamp Rail_V1:10
- Flush:286: 1324_Clamp Rail_V1:9 ↔ 1324_Clamp Rail_V1:12
- Flush:287: 1324_Clamp Rail_V1:11 ↔ 1324_Clamp Rail_V1:14
- Flush:288: 1323_Clamp Holder Pin_V1:8 ↔ 1323_Clamp Holder Pin_V1:10
- Flush:289: 1323_Clamp Holder Pin_V1:10 ↔ 1323_Clamp Holder Pin_V1:12
- Flush:290: 1323_Clamp Holder Pin_V1:12 ↔ 1323_Clamp Holder Pin_V1:14
- Mate:348: 1311_Former Top_V1:1 ↔ 1324_Clamp Rail_V1:8
- Mate:349: 1311_Former Top_V1:1 ↔ 1324_Clamp Rail_V1:8
- Mate:350: 1311_Former Top_V1:1 ↔ 1324_Clamp Rail_V1:8
- Mate:351: 1311_Former Top_V1:1 ↔ 1324_Clamp Rail_V1:9
- Mate:352: 1311_Former Top_V1:1 ↔ 1324_Clamp Rail_V1:12
- Mate:353: 1311_Former Top_V1:1 ↔ 1324_Clamp Rail_V1:14
- Flush:291: 1323_Clamp Holder Pin_V1:4 ↔ 1323_Clamp Holder Pin_V1:8
- Mate:354: 1231_Spool Shaft_V1:1 ↔ 1240_Wire Spool and Wire:1
- Mate:355: 1240_Wire Spool and Wire:1 ↔ 1234_Spool Plate_V1:1
- Mate:356: 1240_Wire Spool and Wire:1 ↔ 1234_Spool Plate_V1:2
- Angle:34 (0 deg): 1240_Wire Spool and Wire:1 ↔ 1234_Spool Plate_V1:2
- Flush:292: 1219_Middle Roller_V1:1 ↔ 1240_Wire Spool and Wire:1
- Flush:293: 1234_Spool Plate_V1:1 ↔ 1234_Spool Plate_V1:2
- Mate:357: 1240_Wire Spool and Wire:1 ↔ 1240x_Wire Depiction_V1:1
- Mate:358: 1240_Wire Spool and Wire:1 ↔ 1240x_Wire Depiction_V1:1
- Angle:35 (0 deg): 1240x_Wire Depiction_V1:1
- Mate:359: 1240_Wire Spool and Wire:1 ↔ 1240x_Wire Depiction_V1:1
- Angle:36 (12 deg): 1225a_Pinion Collar_V1:1 ↔ frame_1385mm:4
- Angle:37 (-1.5 deg): 1236_Spool Shaft Support Plate_V1:1 ↔ 1234_Spool Plate_V1:1
- Flush:294 (3 mm): 1213_Distal Roller_V1:2 ↔ 1240x_Wire Depiction_V1:1
- Flush:295: 1234_Spool Plate_V1:1 ↔ 1234_Spool Plate_V1:2
- Flush:296: 1234_Spool Plate_V1:1 ↔ 1234_Spool Plate_V1:2
- Mate:360: 1231_Spool Shaft_V1:1 ↔ 1234_Spool Plate_V1:1
## Named parameters: Angle = 5.729578 deg, d366_d365 = 0 mm, d367_d351 = 0 mm, d368_d352 = 0 mm, d369_d353 = 0 mm, d370_d354 = 0 mm, d371_d355 = 0 mm, d372_d356 = 0 mm, d373_d357 = 0 mm, d374_d358 = 0 mm, d375_d359 = 0 mm, d376_d360 = 0 mm, d377_d361 = 0 mm, d378_d362 = 0 mm, d379_d363 = 0 mm, d380_d364 = 0 mm, d381_d185 = 0 mm, d382_d186 = 0 mm, d383_d187 = 3 mm, d384_d343 = 0 mm, d385_d344 = 0 mm, d386_d345 = 0 deg, d387_d346 = 0 mm, d388_d347 = 0 mm, d389_d348 = 0 deg, d390_d349 = 0 mm, d391_d350 = 0 mm, AngToFrame = 0 deg, d399_d395 = 0 mm, d400_d396 = 0 mm, d401_d398 = 45 mm, d402_d365 = 0 mm, d403_d366_d365 = 0 mm, d404_d367_d351 = 0 mm, d405_d368_d352 = 0 mm, d406_d369_d353 = 0 mm, d407_d370_d354 = 0 mm, d408_d371_d355 = 0 mm, d409_d372_d356 = 0 mm, d410_d373_d357 = 0 mm, d411_d374_d358 = 0 mm, d412_d375_d359 = 0 mm, d413_d376_d360 = 0 mm, d414_d377_d361 = 0 mm, d415_d378_d362 = 0 mm, d416_d379_d363 = 0 mm, d417_d380_d364 = 0 mm, d418_d381_d185 = 0 mm, d419_d382_d186 = 0 mm, d420_d383_d187 = 3 mm, d421_d384_d343 = 0 mm, d422_d385_d344 = 0 mm, d423_d386_d345 = 0 deg, d424_d387_d346 = 0 mm, d425_d388_d347 = 0 mm, d426_d389_d348 = 0 deg, d427_d390_d349 = 0 mm, d428_d391_d350 = 0 mm, d429_d394 = 0 mm, d430_d351 = 0 mm, d431_d352 = 0 mm, d432_d353 = 0 mm, d433_d354 = 0 mm, d434_d355 = 0 mm, d435_d356 = 0 mm, d436_d357 = 0 mm, d437_d358 = 0 mm, d438_d359 = 0 mm, d439_d360 = 0 mm, d440_d361 = 0 mm, d441_d362 = 0 mm, d442_d363 = 0 mm, d443_d364 = 0 mm, d444_d183 = 45 mm, d445_d184 = 0.5 mm, d446_d185 = 0 mm, d447_d186 = 0 mm, d448_d187 = 3 mm, d449_d343 = 0 mm, d450_d344 = 0 mm, d451_d345 = 0 deg, d452_d346 = 0 mm, d453_d347 = 0 mm, d454_d348 = 0 deg, d455_d349 = 0 mm, d456_d350 = 0 mm, d467_d399_d395 = 0 mm, d468_d400_d396 = 0 mm, d469_d401_d398 = 45 mm, d470_d402_d365 = 0 mm, d471_d403_d366_d365 = 0 mm, d472_d404_d367_d351 = 0 mm, d473_d405_d368_d352 = 0 mm, d474_d406_d369_d353 = 0 mm, d475_d407_d370_d354 = 0 mm, d476_d408_d371_d355 = 0 mm, d477_d409_d372_d356 = 0 mm, d478_d410_d373_d357 = 0 mm, d479_d411_d374_d358 = 0 mm, d480_d412_d375_d359 = 0 mm, d481_d413_d376_d360 = 0 mm, d482_d414_d377_d361 = 0 mm, d483_d415_d378_d362 = 0 mm, d484_d416_d379_d363 = 0 mm, d485_d417_d380_d364 = 0 mm, d486_d418_d381_d185 = 0 mm, d487_d419_d382_d186 = 0 mm, d488_d420_d383_d187 = 3 mm, d489_d421_d384_d343 = 0 mm, d490_d422_d385_d344 = 0 mm, d491_d423_d386_d345 = 0 deg, d492_d424_d387_d346 = 0 mm, d493_d425_d388_d347 = 0 mm, d494_d426_d389_d348 = 0 deg, d495_d427_d390_d349 = 0 mm, d496_d428_d391_d350 = 0 mm, d497_d429_d394 = 0 mm, d498_d430_d351 = 0 mm, d499_d431_d352 = 0 mm, d500_d432_d353 = 0 mm, d501_d433_d354 = 0 mm, d502_d434_d355 = 0 mm, d503_d435_d356 = 0 mm, d504_d436_d357 = 0 mm, d505_d437_d358 = 0 mm, d506_d438_d359 = 0 mm, d507_d439_d360 = 0 mm, d508_d440_d361 = 0 mm, d509_d441_d362 = 0 mm, d510_d442_d363 = 0 mm, d511_d443_d364 = 0 mm, d512_d444_d183 = 45 mm, d513_d445_d184 = 0.5 mm, d514_d446_d185 = 0 mm, d515_d447_d186 = 0 mm, d516_d448_d187 = 3 mm, d517_d449_d343 = 0 mm, d518_d450_d344 = 0 mm, d519_d451_d345 = 0 deg, d520_d452_d346 = 0 mm, d521_d453_d347 = 0 mm, d522_d454_d348 = 0 deg, d523_d455_d349 = 0 mm, d524_d456_d350 = 0 mm, d525_d461 = 0 mm, d526_d464 = 0 mm, d527_d465 = 0 mm, d528_d458 = 0 mm, d529_d459 = 0 mm, d530_d460 = 0 mm, d535_d399_d395 = 0 mm, d536_d400_d396 = 0 mm, d537_d401_d398 = 45 mm, d538_d402_d365 = 0 mm, d539_d403_d366_d365 = 0 mm, d540_d404_d367_d351 = 0 mm, d541_d405_d368_d352 = 0 mm, d542_d406_d369_d353 = 0 mm, d543_d407_d370_d354 = 0 mm, d544_d408_d371_d355 = 0 mm, d545_d409_d372_d356 = 0 mm, d546_d410_d373_d357 = 0 mm, d547_d411_d374_d358 = 0 mm, d548_d412_d375_d359 = 0 mm, d549_d413_d376_d360 = 0 mm, d550_d414_d377_d361 = 0 mm, d551_d415_d378_d362 = 0 mm, d552_d416_d379_d363 = 0 mm, d553_d417_d380_d364 = 0 mm, d554_d418_d381_d185 = 0 mm, d555_d419_d382_d186 = 0 mm, d556_d420_d383_d187 = 3 mm, d557_d421_d384_d343 = 0 mm, d558_d422_d385_d344 = 0 mm, d559_d423_d386_d345 = 0 deg, d560_d424_d387_d346 = 0 mm, d561_d425_d388_d347 = 0 mm, d562_d426_d389_d348 = 0 deg, d563_d427_d390_d349 = 0 mm, d564_d428_d391_d350 = 0 mm, d565_d429_d394 = 0 mm, d566_d430_d351 = 0 mm, d567_d431_d352 = 0 mm, d568_d432_d353 = 0 mm, d569_d433_d354 = 0 mm, d570_d434_d355 = 0 mm, d571_d435_d356 = 0 mm, d572_d436_d357 = 0 mm, d573_d437_d358 = 0 mm, d574_d438_d359 = 0 mm, d575_d439_d360 = 0 mm, d576_d440_d361 = 0 mm, d577_d441_d362 = 0 mm, d578_d442_d363 = 0 mm, d579_d443_d364 = 0 mm, d580_d444_d183 = 45 mm, d581_d445_d184 = 0.5 mm, d582_d446_d185 = 0 mm, d583_d447_d186 = 0 mm, d584_d448_d187 = 3 mm, d585_d449_d343 = 0 mm, d586_d450_d344 = 0 mm, d587_d451_d345 = 0 deg, d588_d452_d346 = 0 mm, d589_d453_d347 = 0 mm, d590_d454_d348 = 0 deg, d591_d455_d349 = 0 mm, d592_d456_d350 = 0 mm, d593_d461 = 0 mm, d594_d464 = 0 mm, d595_d465 = 0 mm, d596_d458 = 0 mm, d597_d459 = 0 mm, d598_d460 = 0 mm, d599_d399_d395 = 0 mm, d600_d400_d396 = 0 mm, d601_d401_d398 = 45 mm, d602_d402_d365 = 0 mm, d603_d403_d366_d365 = 0 mm, d604_d404_d367_d351 = 0 mm, d605_d405_d368_d352 = 0 mm, d606_d406_d369_d353 = 0 mm, d607_d407_d370_d354 = 0 mm, d608_d408_d371_d355 = 0 mm, d609_d409_d372_d356 = 0 mm, d610_d410_d373_d357 = 0 mm, d611_d411_d374_d358 = 0 mm, d612_d412_d375_d359 = 0 mm, d613_d413_d376_d360 = 0 mm, d614_d414_d377_d361 = 0 mm, d615_d415_d378_d362 = 0 mm, d616_d416_d379_d363 = 0 mm, d617_d417_d380_d364 = 0 mm, d618_d418_d381_d185 = 0 mm, d619_d419_d382_d186 = 0 mm, d620_d420_d383_d187 = 3 mm, d621_d421_d384_d343 = 0 mm, d622_d422_d385_d344 = 0 mm, d623_d423_d386_d345 = 0 deg, d624_d424_d387_d346 = 0 mm, d625_d425_d388_d347 = 0 mm, d626_d426_d389_d348 = 0 deg, d627_d427_d390_d349 = 0 mm, d628_d428_d391_d350 = 0 mm, d629_d429_d394 = 0 mm, d630_d430_d351 = 0 mm, d631_d431_d352 = 0 mm, d632_d432_d353 = 0 mm, d633_d433_d354 = 0 mm, d634_d434_d355 = 0 mm, d635_d435_d356 = 0 mm, d636_d436_d357 = 0 mm, d637_d437_d358 = 0 mm, d638_d438_d359 = 0 mm, d639_d439_d360 = 0 mm, d640_d440_d361 = 0 mm, d641_d441_d362 = 0 mm, d642_d442_d363 = 0 mm, d643_d443_d364 = 0 mm, d644_d444_d183 = 45 mm, d645_d445_d184 = 0.5 mm, d646_d446_d185 = 0 mm, d647_d447_d186 = 0 mm, d648_d448_d187 = 3 mm, d649_d449_d343 = 0 mm, d650_d450_d344 = 0 mm, d651_d451_d345 = 0 deg, d652_d452_d346 = 0 mm, d653_d453_d347 = 0 mm, d654_d454_d348 = 0 deg, d655_d455_d349 = 0 mm, d656_d456_d350 = 0 mm, d657_d461 = 0 mm, d658_d464 = 0 mm, d659_d465 = 0 mm, d660_d458 = 0 mm, d661_d459 = 0 mm, d662_d460 = 0 mm, d663_d399_d395 = 0 mm, d664_d400_d396 = 0 mm, d665_d401_d398 = 45 mm, d666_d402_d365 = 0 mm, d667_d403_d366_d365 = 0 mm, d668_d404_d367_d351 = 0 mm, d669_d405_d368_d352 = 0 mm, d670_d406_d369_d353 = 0 mm, d671_d407_d370_d354 = 0 mm, d672_d408_d371_d355 = 0 mm, d673_d409_d372_d356 = 0 mm, d674_d410_d373_d357 = 0 mm, d675_d411_d374_d358 = 0 mm, d676_d412_d375_d359 = 0 mm, d677_d413_d376_d360 = 0 mm, d678_d414_d377_d361 = 0 mm, d679_d415_d378_d362 = 0 mm, d680_d416_d379_d363 = 0 mm, d681_d417_d380_d364 = 0 mm, d682_d418_d381_d185 = 0 mm, d683_d419_d382_d186 = 0 mm, d684_d420_d383_d187 = 3 mm, d685_d421_d384_d343 = 0 mm, d686_d422_d385_d344 = 0 mm, d687_d423_d386_d345 = 0 deg, d688_d424_d387_d346 = 0 mm, d689_d425_d388_d347 = 0 mm, d690_d426_d389_d348 = 0 deg, d691_d427_d390_d349 = 0 mm, d692_d428_d391_d350 = 0 mm, d693_d429_d394 = 0 mm, d694_d430_d351 = 0 mm, d695_d431_d352 = 0 mm, d696_d432_d353 = 0 mm, d697_d433_d354 = 0 mm, d698_d434_d355 = 0 mm, d699_d435_d356 = 0 mm, d700_d436_d357 = 0 mm, d701_d437_d358 = 0 mm, d702_d438_d359 = 0 mm, d703_d439_d360 = 0 mm, d704_d440_d361 = 0 mm, d705_d441_d362 = 0 mm, d706_d442_d363 = 0 mm, d707_d443_d364 = 0 mm, d708_d444_d183 = 45 mm, d709_d445_d184 = 0.5 mm, d710_d446_d185 = 0 mm, d711_d447_d186 = 0 mm, d712_d448_d187 = 3 mm, d713_d449_d343 = 0 mm, d714_d450_d344 = 0 mm, d715_d451_d345 = 0 deg, d716_d452_d346 = 0 mm, d717_d453_d347 = 0 mm, d718_d454_d348 = 0 deg, d719_d455_d349 = 0 mm, d720_d456_d350 = 0 mm, d721_d461 = 0 mm, d722_d464 = 0 mm, d723_d465 = 0 mm, d724_d458 = 0 mm, d725_d459 = 0 mm, d726_d460 = 0 mm, d727_d399_d395 = 0 mm, d728_d400_d396 = 0 mm, d729_d401_d398 = 45 mm, d730_d402_d365 = 0 mm, d731_d403_d366_d365 = 0 mm, d732_d404_d367_d351 = 0 mm, d733_d405_d368_d352 = 0 mm, d734_d406_d369_d353 = 0 mm, d735_d407_d370_d354 = 0 mm, d736_d408_d371_d355 = 0 mm, d737_d409_d372_d356 = 0 mm, d738_d410_d373_d357 = 0 mm, d739_d411_d374_d358 = 0 mm, d740_d412_d375_d359 = 0 mm, d741_d413_d376_d360 = 0 mm, d742_d414_d377_d361 = 0 mm, d743_d415_d378_d362 = 0 mm, d744_d416_d379_d363 = 0 mm, d745_d417_d380_d364 = 0 mm, d746_d418_d381_d185 = 0 mm, d747_d419_d382_d186 = 0 mm, d748_d420_d383_d187 = 3 mm, d749_d421_d384_d343 = 0 mm, d750_d422_d385_d344 = 0 mm, d751_d423_d386_d345 = 0 deg, d752_d424_d387_d346 = 0 mm, d753_d425_d388_d347 = 0 mm, d754_d426_d389_d348 = 0 deg, d755_d427_d390_d349 = 0 mm, d756_d428_d391_d350 = 0 mm, d757_d429_d394 = 0 mm, d758_d430_d351 = 0 mm, d759_d431_d352 = 0 mm, d760_d432_d353 = 0 mm, d761_d433_d354 = 0 mm, d762_d434_d355 = 0 mm, d763_d435_d356 = 0 mm, d764_d436_d357 = 0 mm, d765_d437_d358 = 0 mm, d766_d438_d359 = 0 mm, d767_d439_d360 = 0 mm, d768_d440_d361 = 0 mm, d769_d441_d362 = 0 mm, d770_d442_d363 = 0 mm, d771_d443_d364 = 0 mm, d772_d444_d183 = 45 mm, d773_d445_d184 = 0.5 mm, d774_d446_d185 = 0 mm, d775_d447_d186 = 0 mm, d776_d448_d187 = 3 mm, d777_d449_d343 = 0 mm, d778_d450_d344 = 0 mm, d779_d451_d345 = 0 deg, d780_d452_d346 = 0 mm, d781_d453_d347 = 0 mm, d782_d454_d348 = 0 deg, d783_d455_d349 = 0 mm, d784_d456_d350 = 0 mm, d785_d461 = 0 mm, d786_d464 = 0 mm, d787_d465 = 0 mm, d788_d458 = 0 mm, d789_d459 = 0 mm, d790_d460 = 0 mm, FormerAngToFrame = 1 deg, PinionAngle = 12 deg
